# Autodesk Inventor assembly: Ensamble
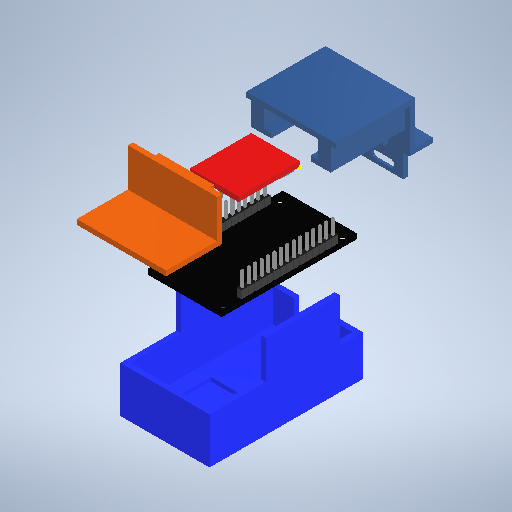
[picture p0: Inventor's stored thumbnail of the model, 512x512]
Saved by Autodesk Inventor 2025.1 (Build 291241020, 241B)
## iProperties
Created: 2024-08-30
Part Number: Ensamble
Document SubType Name: Assembly
Designer: andre
Author: andre
## Documents named in this file (6)
- C:\Users\andre\OneDrive_Personal\OneDrive\UCR\TCU\Diseño\Ensamble.iam
- C:\Users\andre\OneDrive_Personal\OneDrive\UCR\TCU\Diseño\Carcaza.ipt
- C:\Users\andre\OneDrive_Personal\OneDrive\UCR\TCU\Diseño\ESP32_DevBoard.ipt
- C:\Users\andre\OneDrive_Personal\OneDrive\UCR\TCU\Diseño\Circuit.ipt
- C:\Users\andre\OneDrive_Personal\OneDrive\UCR\TCU\Diseño\TapaCarcaza.ipt
- C:\Users\andre\OneDrive_Personal\OneDrive\UCR\TCU\Diseño\TapaTrasera.ipt
## Components (5 placed, 5 different names)
1. Carcaza:1 — Mate:3
2. ESP32_DevBoard:1 — Mate:3
3. Circuit:1 — Mate:5, Mate:13
4. TapaCarcaza:1 — Mate:5, Mate:11, Mate:12, Mate:13
5. TapaTrasera:1 — Mate:11, Mate:12
## Relationships (5: Mate 5)
- Mate:3 (1 mm): Carcaza:1 ↔ ESP32_DevBoard:1
- Mate:5: Circuit:1 ↔ TapaCarcaza:1
- Mate:11 (-5 mm): TapaCarcaza:1 ↔ TapaTrasera:1
- Mate:12: TapaCarcaza:1 ↔ TapaTrasera:1
- Mate:13 (1.25 mm): Circuit:1 ↔ TapaCarcaza:1
## Named parameters: w = 2 mm
